# Autodesk Inventor assembly: Assembly1
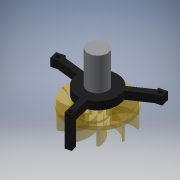
[picture p0: Inventor's stored thumbnail of the model, 180x180]
Saved by Autodesk Inventor 2016 (Build 200138000, 138)
## iProperties
Created: 2016-12-03
Part Number: Assembly1
Material: 一般
Document SubType Name: Assembly
Designer: kota
Author: kota
## Documents named in this file (4)
- C:\Users\B4_Ohno\Dropbox\AliCe\MicroMouse2016\Assembly1.iam
- C:\Users\B4_Ohno\Dropbox\AliCe\MicroMouse2016\s_fan.ipt
- C:\Users\B4_Ohno\Dropbox\AliCe\MicroMouse2016\s_mount.ipt
- C:\Users\B4_Ohno\Dropbox\AliCe\MicroMouse2016\s_motor.ipt
## Components (3 placed, 3 different names)
1. s_motor:1 — リジッド:1, リジッド:2
2. s_fan:1 — リジッド:2
3. s_mount:1 — リジッド:1
## Relationships (2: WeldJoint 2)
- リジッド:1 [WeldJoint]: s_motor:1 ↔ s_mount:1
- リジッド:2 [WeldJoint]: s_motor:1 ↔ s_fan:1
